# Autodesk Inventor assembly: LPTL_ASSEMBLY WITH SUPPORT
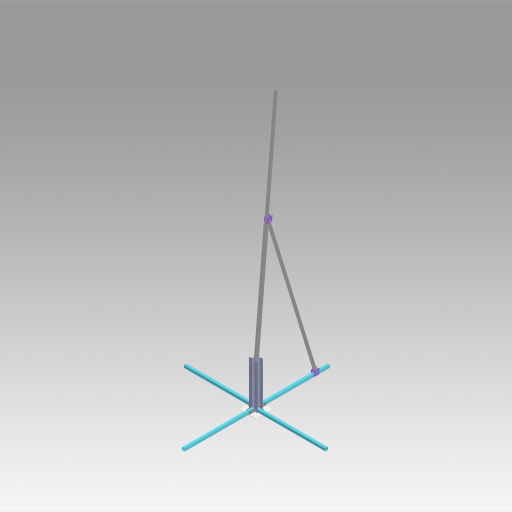
[picture p0: Inventor's stored thumbnail of the model, 512x512]
Saved by Autodesk Inventor 2023 (Build 270158000, 158)
## iProperties
Created: 2025-04-16
Part Number: LPTL_ASSEMBLY WITH SUPPORT
Document SubType Name: Assembly
Designer: NELLY NDUNG'U
Author: NELLY NDUNG'U
## Documents named in this file (14)
- N:\NAKUJA\CAD FILES\AIRFRAME\LP003\LPTL_ASSEMBLY WITH SUPPORT.iam
- N:\NAKUJA\CAD FILES\AIRFRAME\LP003\BASE_ASSEMBLY.iam
- N:\NAKUJA\CAD FILES\AIRFRAME\LP003\TL_50_40.iam
- N:\NAKUJA\CAD FILES\AIRFRAME\LP003\SUPPORT ATTACHMENT.ipt
- N:\NAKUJA\CAD FILES\AIRFRAME\LP003\ENFORCEMENT.iam
- C:\Users\User\Documents\Inventor\Content Center Files\R2023\en-US\ANSI B18.2.3.5M\ANSI B18.2.3.5M - M16 x 2 x 65.ipt
- C:\Users\User\Documents\Inventor\Content Center Files\R2023\en-US\ANSI B18.2.3.5M\ANSI B18.2.3.5M - M16 x 2 x 80.ipt
- C:\Users\User\Documents\Inventor\Content Center Files\R2023\en-US\ANSI B 18.2.4.1 M(1)\ANSI B 18.2.4.1 M - M16 x 2Style 1.ipt
- N:\NAKUJA\CAD FILES\AIRFRAME\LP003\LPTL_ASSEMBLY WITH SUPPORT\AIP\FEA\f1b1ifc8w.fins
- N:\NAKUJA\CAD FILES\AIRFRAME\LP003\LPTL_ASSEMBLY WITH SUPPORT\AIP\FEA\f1b1ifc8w.fsat
- N:\NAKUJA\CAD FILES\AIRFRAME\LP003\LPTL_ASSEMBLY WITH SUPPORT\AIP\FEA\f1b1ifc8w.ftes
- N:\NAKUJA\CAD FILES\AIRFRAME\LP003\LPTL_ASSEMBLY WITH SUPPORT\AIP\FEA\f1b1ifc9s.fwiz
- N:\NAKUJA\CAD FILES\AIRFRAME\LP003\LPTL_ASSEMBLY WITH SUPPORT\AIP\FEA\f1b1ifdfk.fmsh
- N:\NAKUJA\CAD FILES\AIRFRAME\LP003\LPTL_ASSEMBLY WITH SUPPORT\AIP\FEA\f1b1ifdfl.fres
## Components (17 placed, 7 different names)
1. BASE_ASSEMBLY:1 [sub-assembly] — Angle:1, Mate:1, Mate:2, Mate:3, Mate:5, Angle:2, Mate:8, Mate:11, Mate:12, Flush:3, Flush:4, Mate:13, Mate:14, Insert:2, Insert:3, Insert:4, Insert:7, Insert:8, Insert:9
2. TL_50_40:1 [sub-assembly] — Angle:1, Mate:1, Mate:2, Mate:3, Flush:1, Mate:4, Flush:2, Mate:6, Mate:9
3. SUPPORT ATTACHMENT:1 — Flush:1, Mate:4, Mate:5, Mate:7, Insert:6
4. SUPPORT ATTACHMENT:2 — Flush:2, Mate:6, Mate:7, Mate:10, Insert:1
5. ENFORCEMENT:1 [sub-assembly] — Angle:2, Mate:8, Mate:9, Mate:10
6. SUPPORT ATTACHMENT:3 — Mate:11, Flush:3, Mate:13, Insert:10
7. SUPPORT ATTACHMENT:4 — Mate:12, Flush:4, Mate:14, Insert:5
8. Hex Bolt - Metric M16 x 2 x 65:1 — Insert:1
9. Hex Bolt - Metric M16 x 2 x 80:1 — Insert:2
10. Hex Bolt - Metric M16 x 2 x 80:2 — Insert:3
11. Hex Bolt - Metric M16 x 2 x 80:3 — Insert:4
12. Hex Bolt - Metric M16 x 2 x 65:2 — Insert:5
13. Hex Nut Metric M16 x 2:1 — Insert:6
14. Hex Nut Metric M16 x 2:2 — Insert:7
15. Hex Nut Metric M16 x 2:3 — Insert:8
16. Hex Nut Metric M16 x 2:4 — Insert:9
17. Hex Nut Metric M16 x 2:5 — Insert:10
## Relationships (30: Mate 14, Insert 10, Flush 4, Angle 2)
- Angle:1 (85 deg): BASE_ASSEMBLY:1 ↔ TL_50_40:1
- Mate:1 (-300 mm): BASE_ASSEMBLY:1 ↔ TL_50_40:1
- Mate:2: BASE_ASSEMBLY:1 ↔ TL_50_40:1
- Mate:3 (-8 mm): BASE_ASSEMBLY:1 ↔ TL_50_40:1
- Flush:1: TL_50_40:1 ↔ SUPPORT ATTACHMENT:1
- Mate:4: TL_50_40:1 ↔ SUPPORT ATTACHMENT:1
- Mate:5 (2770 mm): BASE_ASSEMBLY:1 ↔ SUPPORT ATTACHMENT:1
- Flush:2: TL_50_40:1 ↔ SUPPORT ATTACHMENT:2
- Mate:6: TL_50_40:1 ↔ SUPPORT ATTACHMENT:2
- Mate:7: SUPPORT ATTACHMENT:1 ↔ SUPPORT ATTACHMENT:2
- Angle:2 (73 deg): BASE_ASSEMBLY:1 ↔ ENFORCEMENT:1
- Mate:8: BASE_ASSEMBLY:1 ↔ ENFORCEMENT:1
- Mate:9: TL_50_40:1 ↔ ENFORCEMENT:1
- Mate:10: SUPPORT ATTACHMENT:2 ↔ ENFORCEMENT:1
- Mate:11 (-5 mm): BASE_ASSEMBLY:1 ↔ SUPPORT ATTACHMENT:3
- Mate:12 (-5 mm): BASE_ASSEMBLY:1 ↔ SUPPORT ATTACHMENT:4
- Flush:3: BASE_ASSEMBLY:1 ↔ SUPPORT ATTACHMENT:3
- Flush:4: BASE_ASSEMBLY:1 ↔ SUPPORT ATTACHMENT:4
- Mate:13 (960 mm): BASE_ASSEMBLY:1 ↔ SUPPORT ATTACHMENT:3
- Mate:14 (960 mm): BASE_ASSEMBLY:1 ↔ SUPPORT ATTACHMENT:4
- Insert:1: SUPPORT ATTACHMENT:2 ↔ Hex Bolt - Metric M16 x 2 x 65:1
- Insert:2: BASE_ASSEMBLY:1 ↔ Hex Bolt - Metric M16 x 2 x 80:1
- Insert:3: BASE_ASSEMBLY:1 ↔ Hex Bolt - Metric M16 x 2 x 80:2
- Insert:4: BASE_ASSEMBLY:1 ↔ Hex Bolt - Metric M16 x 2 x 80:3
- Insert:5: SUPPORT ATTACHMENT:4 ↔ Hex Bolt - Metric M16 x 2 x 65:2
- Insert:6: SUPPORT ATTACHMENT:1 ↔ Hex Nut Metric M16 x 2:1
- Insert:7: BASE_ASSEMBLY:1 ↔ Hex Nut Metric M16 x 2:2
- Insert:8: BASE_ASSEMBLY:1 ↔ Hex Nut Metric M16 x 2:3
- Insert:9: BASE_ASSEMBLY:1 ↔ Hex Nut Metric M16 x 2:4
- Insert:10: SUPPORT ATTACHMENT:3 ↔ Hex Nut Metric M16 x 2:5
## Named parameters: sa_0 = 30000
note: some values were not read from the file. Shown as the stored number, unit unknown: "sa_0".
